# Autodesk Inventor assembly: ToASI-6
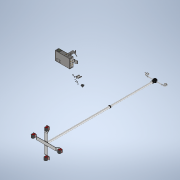
[picture p0: Inventor's stored thumbnail of the model, 180x180]
Saved by Autodesk Inventor 2020.3 (Build 243373000, 373)
## iProperties
Created: 2020-08-01
Part Number: ToASI-6
Document SubType Name: Assembly
Designer: Bruno
Author: Bruno
## Documents named in this file (10)
- C:\Users\Bruno\Desktop\Github\CAD\Inventor\For ASI\ToASI-6.iam
- C:\Users\Bruno\Desktop\Github\CAD\Inventor\For ASI\ToASI-4.iam
- C:\Users\Bruno\Desktop\Github\CAD\Inventor\Heater-Box\Glass vase _ flow meter fixer\Glass fixer plate.ipt
- C:\Users\Bruno\Desktop\Github\CAD\Inventor\Heater-Box\Glass vase _ flow meter fixer\DIN912 M4x0.7x10-8.8 socket head screw.ipt
- C:\Users\Bruno\Desktop\Github\CAD\Inventor\Heater-Box\IV stand fixer\Box-iv stand Connector.ipt
- C:\Users\Bruno\Desktop\Github\CAD\Inventor\Heater-Box\IV stand fixer\DIN912 M4x0.7x10-8.8 socket head screw.ipt
- C:\Users\Bruno\Desktop\Github\CAD\Inventor\Heater-Box\IV stand fixer\Split Washer DIN127B D4.ipt
- C:\Users\Bruno\Desktop\Github\CAD\Inventor\Heater-Box\IV stand fixer\DIN934-M4 nut.ipt
- C:\Users\Bruno\Desktop\Github\CAD\Inventor\Heater-Box\IV stand fixer\Star Knob 1-4UNC.ipt
- C:\Users\Bruno\Desktop\Github\CAD\Inventor\Auxiliary Components\IV Stand.ipt
## Components (18 placed, 8 different names)
1. ToASI-4:1 [sub-assembly] — Cylindrical:1, Cylindrical:4
2. Glass fixer plate:1 — Cylindrical:1, Cylindrical:2, Cylindrical:3
3. DIN912 M4x0.7x10-8.8 socket head screw:1 — Cylindrical:3
4. DIN912 M4x0.7x10-8.8 socket head screw:2 — Cylindrical:2
5. Box-iv stand Connector:1 — Cylindrical:4
6. Box-iv stand Connector:2
7. DIN912 M4x0.7x10-8.8 socket head screw:3
8. DIN912 M4x0.7x10-8.8 socket head screw:4
9. DIN912 M4x0.7x10-8.8 socket head screw:5
10. DIN912 M4x0.7x10-8.8 socket head screw:6
11. DIN912 M4x0.7x10-8.8 socket head screw:7
12. DIN912 M4x0.7x10-8.8 socket head screw:8
13. Split Washer DIN127B D4:1
14. Split Washer DIN127B D4:2
15. DIN934-M4 nut:1
16. DIN934-M4 nut:2
17. Star Knob 1-4UNC:1
18. IV Stand:1
## Relationships (4: CylindricalJoint 4)
- Cylindrical:1: ToASI-4:1 ↔ Glass fixer plate:1
- Cylindrical:2: Glass fixer plate:1 ↔ DIN912 M4x0.7x10-8.8 socket head screw:2
- Cylindrical:3: Glass fixer plate:1 ↔ DIN912 M4x0.7x10-8.8 socket head screw:1
- Cylindrical:4: ToASI-4:1 ↔ Box-iv stand Connector:1
